# Autodesk Inventor assembly: s-assy-link2
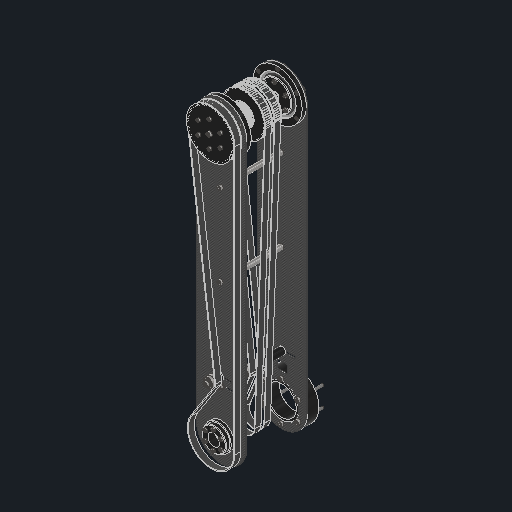
[picture p0: Inventor's stored thumbnail of the model, 512x512]
Saved by Autodesk Inventor 2022 (Build 260153000, 153)
## iProperties
Created: 2021-07-17
Part Number: s-assy-link2
Document SubType Name: Assembly
Designer: yuta0
Mass: 1448.61 g
Surface Area: 6046.34 cm^2
Volume: 815.942 cm^3
Density: 1.77539 g/cm^3
Author: yuta0
## Documents named in this file (25)
- C:\Users\yuta0\Documents\GitHub\catchrobo_hardware\assy-robot\s-assy-link2.iam
- C:\Users\yuta0\Documents\GitHub\catchrobo_hardware\assy-robot\carbon_plate3.ipt
- C:\Users\yuta0\Documents\GitHub\catchrobo_hardware\assy-robot\base30.ipt
- C:\Users\yuta0\Documents\GitHub\catchrobo_hardware\assy-robot\carbon_plate2.ipt
- C:\Users\yuta0\Documents\GitHub\catchrobo_hardware\assy-robot\s-assy-link2-bearing.iam
- C:\Users\yuta0\Documents\GitHub\catchrobo_hardware\assy-robot\s-assy-pulley-j3.iam
- C:\Users\yuta0\Documents\GitHub\catchrobo_hardware\assy-robot\base14.ipt
- C:\Users\yuta0\Documents\GitHub\catchrobo_hardware\assy-robot\base3.ipt
- C:\Users\yuta0\Documents\GitHub\catchrobo_hardware\assy-robot\CB3-20.ipt
- C:\Users\yuta0\Documents\GitHub\catchrobo_hardware\assy-robot\belt_1.ipt
- C:\Users\yuta0\Documents\GitHub\catchrobo_hardware\assy-robot\tentioner1.iam
- C:\Users\yuta0\Documents\GitHub\catchrobo_hardware\assy-robot\CB4-40.ipt
- C:\Users\yuta0\Documents\GitHub\catchrobo_hardware\assy-robot\base1.ipt
- C:\Users\yuta0\Documents\GitHub\catchrobo_hardware\assy-robot\belt_2.ipt
- C:\Users\yuta0\Documents\GitHub\catchrobo_hardware\assy-robot\CC-0814-05.ipt
- C:\Users\yuta0\Documents\GitHub\catchrobo_hardware\assy-robot\LBNR3.ipt
- C:\Users\yuta0\Documents\GitHub\catchrobo_hardware\assy-robot\CB3-35.ipt
- C:\Users\yuta0\Documents\GitHub\catchrobo_hardware\assy-robot\s-assy-spacer2.ipt.iam
- C:\Users\yuta0\Documents\GitHub\catchrobo_hardware\assy-robot\s-assy-spacer4.iam
- C:\Users\yuta0\Documents\GitHub\catchrobo_hardware\assy-robot\CBSTNR3-16.ipt
- C:\Users\yuta0\Documents\GitHub\catchrobo_hardware\assy-robot\base18.ipt
- C:\Users\yuta0\Documents\GitHub\catchrobo_hardware\assy-robot\SFHRW8-98-M4-N4.ipt
- C:\Users\yuta0\Documents\GitHub\catchrobo_hardware\assy-robot\CB4-25.ipt
- C:\Users\yuta0\Documents\GitHub\catchrobo_hardware\assy-robot\CB4-10.ipt
- s-assy-spacer2.ipt
## Components (77 placed, 23 different names)
1. carbon_plate3:1 — メイト:2, メイト:3, メイト:23, メイト:155, メイト:157, メイト:169, メイト:170, メイト:259, メイト:277, メイト:278
2. base30:1 — メイト:1, メイト:2, メイト:3
3. carbon_plate2:1 — メイト:21, メイト:26, メイト:158, メイト:173, メイト:174, メイト:235, メイト:264, メイト:273, メイト:274, メイト:275, メイト:276, メイト:280, メイト:281
4. s-assy-link2-bearing:1 [sub-assembly] — メイト:23, メイト:154, メイト:155, メイト:156, メイト:157, メイト:258
5. s-assy-link2-bearing:2 [sub-assembly] — メイト:26, メイト:158, メイト:159, メイト:233, メイト:252, メイト:263
6. s-assy-pulley-j3:1 [sub-assembly] — メイト:77, メイト:78, メイト:80, メイト:186, メイト:217, メイト:288
7. s-assy-pulley-j3:2 [sub-assembly] — メイト:78, メイト:187, メイト:254, メイト:285
8. base14:1 — メイト:77, メイト:159, メイト:183, メイト:232, メイト:252, メイト:261, メイト:267, メイト:270, メイト:271, メイト:294, メイト:295
9. base3:1 — メイト:47, メイト:48, メイト:80, メイト:154, メイト:156, メイト:260, メイト:269, メイト:286, メイト:289, メイト:290, メイト:296, メイト:297
10. base1:1 — メイト:173, メイト:174, メイト:189, メイト:190, メイト:231, メイト:283
11. belt_1:1 — メイト:183, メイト:231, メイト:232, メイト:250
12. belt_2:2 — メイト:187, メイト:190, メイト:279
13. belt_2:1 — メイト:186, メイト:189, メイト:233
14. base34:1 — メイト:217, メイト:254, メイト:292
15. tentioner1:1 [sub-assembly] — メイト:235, メイト:250
16. s-assy-spacer2.ipt:1 [sub-assembly] — メイト:273, メイト:276, メイト:277
17. s-assy-spacer2.ipt:2 [sub-assembly] — メイト:274, メイト:275
18. s-assy-spacer4:1 [sub-assembly] — メイト:278, メイト:279
19. base18:1 — メイト:285, メイト:286, メイト:291
20. base18:2 — メイト:288, メイト:293
21. SFHRW8-98-M4-N4:1 — メイト:289, メイト:290, メイト:291, メイト:292, メイト:293
22. CB4-25:1 — メイト:294, メイト:295
23. CB4-10:1 — メイト:296, メイト:297
24. CB4-40:1 — メイト:169, メイト:170
25. CBSTNR3-16:1 — メイト:280, メイト:281, メイト:282
26. LBNR3:35 — メイト:282, メイト:283
27. CB4-40:2
28. CBSTNR3-16:2
29. LBNR3:36
30. CB4-40:3
31. CBSTNR3-16:3
32. LBNR3:37
33. CB4-40:4
34. CBSTNR3-16:4
35. LBNR3:38
36. CB4-40:5
37. CBSTNR3-16:5
38. LBNR3:39
39. CB4-40:6
40. CBSTNR3-16:6
41. LBNR3:40
42. CB3-35:1 — メイト:270, メイト:271, メイト:272
43. LBNR3:7 — メイト:263, メイト:264
44. LBNR3:13 — メイト:267, メイト:272
45. CB3-20:1 — メイト:47, メイト:48, メイト:268
46. LBNR3:1 — メイト:258, メイト:259
47. LBNR3:14 — メイト:268, メイト:269
48. CB3-35:2
49. LBNR3:15
50. LBNR3:16
51. CB3-20:2
52. LBNR3:17
53. LBNR3:18
54. CB3-35:3
55. LBNR3:19
56. LBNR3:20
57. CB3-20:3
58. LBNR3:21
59. LBNR3:22
60. CB3-35:4
61. LBNR3:23
62. LBNR3:24
63. CB3-20:4
64. LBNR3:25
65. LBNR3:26
66. CB3-35:5
67. LBNR3:27
68. LBNR3:28
69. CB3-20:5
70. LBNR3:29
71. LBNR3:30
72. CB3-35:6
73. LBNR3:31
74. LBNR3:32
75. CB3-20:6
76. LBNR3:33
77. LBNR3:34
## Component patterns: (6 elements, first: CB4-40:1 + CBSTNR3-16:1 + LBNR3:35), (6 elements, first: CB3-35:1 + LBNR3:7 + LBNR3:13 + CB3-20:1 + LBNR3:1 + LBNR3:14)
## Relationships (69: Mate 69)
- メイト:1 [Mate]: base30:1
- メイト:2 [Mate]: carbon_plate3:1 ↔ base30:1
- メイト:3 [Mate]: carbon_plate3:1 ↔ base30:1
- メイト:21 [Mate]: carbon_plate2:1
- メイト:23 [Mate]: carbon_plate3:1 ↔ s-assy-link2-bearing:1
- メイト:26 [Mate]: carbon_plate2:1 ↔ s-assy-link2-bearing:2
- メイト:47 [Mate]: base3:1 ↔ CB3-20:1
- メイト:48 [Mate]: base3:1 ↔ CB3-20:1
- メイト:77 [Mate]: s-assy-pulley-j3:1 ↔ base14:1
- メイト:78 [Mate]: s-assy-pulley-j3:1 ↔ s-assy-pulley-j3:2
- メイト:80 [Mate]: s-assy-pulley-j3:1 ↔ base3:1
- メイト:154 [Mate]: s-assy-link2-bearing:1 ↔ base3:1
- メイト:155 [Mate]: carbon_plate3:1 ↔ s-assy-link2-bearing:1
- メイト:156 [Mate]: s-assy-link2-bearing:1 ↔ base3:1
- メイト:157 [Mate]: carbon_plate3:1 ↔ s-assy-link2-bearing:1
- メイト:158 [Mate]: carbon_plate2:1 ↔ s-assy-link2-bearing:2
- メイト:159 [Mate]: s-assy-link2-bearing:2 ↔ base14:1
- メイト:169 [Mate]: carbon_plate3:1 ↔ CB4-40:1
- メイト:170 [Mate]: carbon_plate3:1 ↔ CB4-40:1
- メイト:173 [Mate]: carbon_plate2:1 ↔ base1:1
- メイト:174 [Mate]: carbon_plate2:1 ↔ base1:1
- メイト:183 [Mate] (0.5 mm): base14:1 ↔ belt_1:1
- メイト:186 [Mate] (0.5 mm): s-assy-pulley-j3:1 ↔ belt_2:1
- メイト:187 [Mate] (0.5 mm): s-assy-pulley-j3:2 ↔ belt_2:2
- メイト:189 [Mate]: base1:1 ↔ belt_2:1
- メイト:190 [Mate]: base1:1 ↔ belt_2:2
- メイト:217 [Mate]: s-assy-pulley-j3:1 ↔ base34:1
- メイト:231 [Mate]: base1:1 ↔ belt_1:1
- メイト:232 [Mate]: base14:1 ↔ belt_1:1
- メイト:233 [Mate]: s-assy-link2-bearing:2 ↔ belt_2:1
- メイト:235 [Mate]: carbon_plate2:1 ↔ tentioner1:1
- メイト:250 [Mate]: belt_1:1 ↔ tentioner1:1
- メイト:252 [Mate]: s-assy-link2-bearing:2 ↔ base14:1
- メイト:254 [Mate]: s-assy-pulley-j3:2 ↔ base34:1
- メイト:258 [Mate]: s-assy-link2-bearing:1 ↔ LBNR3:1
- メイト:259 [Mate]: carbon_plate3:1 ↔ LBNR3:1
- メイト:260 [Mate]: base3:1
- メイト:261 [Mate]: base14:1
- メイト:263 [Mate]: s-assy-link2-bearing:2 ↔ LBNR3:7
- メイト:264 [Mate]: carbon_plate2:1 ↔ LBNR3:7
- メイト:267 [Mate] (2 mm): base14:1 ↔ LBNR3:13
- メイト:268 [Mate]: CB3-20:1 ↔ LBNR3:14
- メイト:269 [Mate] (2 mm): base3:1 ↔ LBNR3:14
- メイト:270 [Mate]: base14:1 ↔ CB3-35:1
- メイト:271 [Mate]: base14:1 ↔ CB3-35:1
- メイト:272 [Mate]: CB3-35:1 ↔ LBNR3:13
- メイト:273 [Mate]: carbon_plate2:1 ↔ s-assy-spacer2.ipt:1
- メイト:274 [Mate]: carbon_plate2:1 ↔ s-assy-spacer2.ipt:2
- メイト:275 [Mate]: carbon_plate2:1 ↔ s-assy-spacer2.ipt:2
- メイト:276 [Mate]: carbon_plate2:1 ↔ s-assy-spacer2.ipt:1
- メイト:277 [Mate]: carbon_plate3:1 ↔ s-assy-spacer2.ipt:1
- メイト:278 [Mate]: carbon_plate3:1 ↔ s-assy-spacer4:1
- メイト:279 [Mate]: belt_2:2 ↔ s-assy-spacer4:1
- メイト:280 [Mate]: carbon_plate2:1 ↔ CBSTNR3-16:1
- メイト:281 [Mate]: carbon_plate2:1 ↔ CBSTNR3-16:1
- メイト:282 [Mate]: CBSTNR3-16:1 ↔ LBNR3:35
- メイト:283 [Mate]: base1:1 ↔ LBNR3:35
- メイト:285 [Mate]: s-assy-pulley-j3:2 ↔ base18:1
- メイト:286 [Mate] (2 mm): base3:1 ↔ base18:1
- メイト:288 [Mate]: s-assy-pulley-j3:1 ↔ base18:2
- メイト:289 [Mate]: base3:1 ↔ SFHRW8-98-M4-N4:1
- メイト:290 [Mate]: base3:1 ↔ SFHRW8-98-M4-N4:1
- メイト:291 [Mate]: base18:1 ↔ SFHRW8-98-M4-N4:1
- メイト:292 [Mate]: base34:1 ↔ SFHRW8-98-M4-N4:1
- メイト:293 [Mate]: base18:2 ↔ SFHRW8-98-M4-N4:1
- メイト:294 [Mate]: base14:1 ↔ CB4-25:1
- メイト:295 [Mate]: base14:1 ↔ CB4-25:1
- メイト:296 [Mate]: base3:1 ↔ CB4-10:1
- メイト:297 [Mate]: base3:1 ↔ CB4-10:1
